# Autodesk Inventor assembly: Cơ cấu gạt cốc
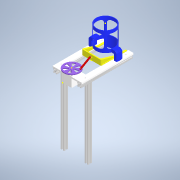
[picture p0: Inventor's stored thumbnail of the model, 180x180]
Saved by Autodesk Inventor 2020 (Build 240168000, 168)
## iProperties
Created: 2022-11-23
Part Number: Cơ cấu gạt cốc
Document SubType Name: Assembly
Designer: ADMIN
_SolveAssemblyDoc: Frame Generator Solve Assembly
_Version: 15.0.0
Author: ADMIN
## Documents named in this file (10)
- D:\Do-an-tot-nghiep\Inventor\Cơ cấu gạt cốc.iam
- D:\Do-an-tot-nghiep\Inventor\Hộp đựng động cơ.ipt
- D:\Do-an-tot-nghiep\Inventor\Khay đựng cốc.ipt
- D:\Do-an-tot-nghiep\Inventor\Khay gạt cốc.ipt
- D:\Do-an-tot-nghiep\Inventor\tay quay.ipt
- C:\Users\ADMIN\OneDrive\Documents\Inventor\Content Center Files\R2020\en-US\ISO 2338(2)\ISO 2338 - 4 h8 x 8.ipt
- D:\Do-an-tot-nghiep\Inventor\step\Assembly1.iam
- D:\Do-an-tot-nghiep\Inventor\trục quay.ipt
- D:\Do-an-tot-nghiep\Inventor\Khung đỡ gạt cốc.ipt
- D:\Do-an-tot-nghiep\Inventor\Cơ cấu gạt cốc\Frame\Frame 1670578973585.iam
## Components (11 placed, 9 different names)
1. Hộp đựng động cơ:1 — Mate:1, Mate:6, Mate:7, Mate:8, Mate:13, Flush:4, Mate:14, Mate:15, Mate:21, Flush:7, Flush:8, Mate:22, Flush:9, Flush:10, Flush:11
2. Khay đựng cốc:1 — Mate:1, Mate:14, Mate:15
3. Khay gạt cốc:1 — Mate:3, Mate:4, Mate:13, Flush:4
4. tay quay:1 — Mate:3, Mate:4, Mate:16, Mate:17, Mate:18, Flush:5, Mate:20, Flush:6
5. Assembly1:1 [sub-assembly] — Mate:6, Mate:7, Mate:8, Mate:9
6. trục quay:1 — Mate:9, Mate:16, Mate:17
7. ISO 2338 4 h8 x 8:2 — Mate:18, Flush:5
8. ISO 2338 4 h8 x 8:3 — Mate:20, Flush:6
9. Khung đỡ gạt cốc:1
10. Frame 1670578973585:1 [sub-assembly] — Mate:21, Flush:7, Flush:9
11. Frame 1670578973585:2 [sub-assembly] — Flush:8, Mate:22, Flush:10, Flush:11
## Relationships (24: Mate 16, Flush 8)
- Mate:1: Hộp đựng động cơ:1 ↔ Khay đựng cốc:1
- Mate:3: Khay gạt cốc:1 ↔ tay quay:1
- Mate:4: Khay gạt cốc:1 ↔ tay quay:1
- Mate:6: Hộp đựng động cơ:1 ↔ Assembly1:1
- Mate:7: Hộp đựng động cơ:1 ↔ Assembly1:1
- Mate:8: Hộp đựng động cơ:1 ↔ Assembly1:1
- Mate:9: Assembly1:1 ↔ trục quay:1
- Mate:13: Hộp đựng động cơ:1 ↔ Khay gạt cốc:1
- Flush:4 (50 mm): Hộp đựng động cơ:1 ↔ Khay gạt cốc:1
- Mate:14: Hộp đựng động cơ:1 ↔ Khay đựng cốc:1
- Mate:15: Hộp đựng động cơ:1 ↔ Khay đựng cốc:1
- Mate:16: tay quay:1 ↔ trục quay:1
- Mate:17: tay quay:1 ↔ trục quay:1
- Mate:18: tay quay:1 ↔ ISO 2338 4 h8 x 8:2
- Flush:5: tay quay:1 ↔ ISO 2338 4 h8 x 8:2
- Mate:20: tay quay:1 ↔ ISO 2338 4 h8 x 8:3
- Flush:6: tay quay:1 ↔ ISO 2338 4 h8 x 8:3
- Mate:21: Hộp đựng động cơ:1 ↔ Frame 1670578973585:1
- Flush:7: Hộp đựng động cơ:1 ↔ Frame 1670578973585:1
- Flush:8: Hộp đựng động cơ:1 ↔ Frame 1670578973585:2
- Mate:22: Hộp đựng động cơ:1 ↔ Frame 1670578973585:2
- Flush:9 (-4 mm): Hộp đựng động cơ:1 ↔ Frame 1670578973585:1
- Flush:10 (-4 mm): Hộp đựng động cơ:1 ↔ Frame 1670578973585:2
- Flush:11: Hộp đựng động cơ:1 ↔ Frame 1670578973585:2
